# Autodesk Inventor assembly: A103EnsembleChariotCarre
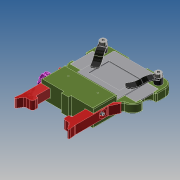
[picture p0: Inventor's stored thumbnail of the model, 180x180]
Saved by Autodesk Inventor 2019 (Build 230136000, 136)
## iProperties
Created: 2016-11-23
Part Number: A103EnsembleChariotCarre
Document SubType Name: Assembly
Designer: serge.amoos
Author: serge.amoos
## Documents named in this file (14)
- Y:\serge.amoos\AAA-FichiersTries\FocalMeasure\A103EnsembleChariotCarre.iam
- Y:\serge.amoos\AAA-FichiersTries\FocalMeasure\P110Poussoir.ipt
- Y:\serge.amoos\AAA-FichiersTries\FocalMeasure\P111Molette.ipt
- Y:\serge.amoos\AAA-FichiersTries\FocalMeasure\P109Ecrou.ipt
- Y:\serge.amoos\AAA-FichiersTries\FocalMeasure\p104levier1.ipt
- Y:\serge.amoos\AAA-FichiersTries\FocalMeasure\p105levier2.ipt
- Y:\serge.amoos\AAA-FichiersTries\FocalMeasure\P103Bielle.ipt
- Y:\serge.amoos\AAA-FichiersTries\FocalMeasure\P113TigeFileteeM3.ipt
- Y:\serge.amoos\AAA-FichiersTries\FocalMeasure\F106EcrouM3.ipt
- Y:\serge.amoos\AAA-FichiersTries\FocalMeasure\F114DiaReseau.ipt
- Y:\serge.amoos\AAA-FichiersTries\FocalMeasure\F115Reseau.ipt
- Y:\serge.amoos\AAA-FichiersTries\FocalMeasure\P124Pince.ipt
- Y:\serge.amoos\AAA-FichiersTries\FocalMeasure\F116VisTcyl6pcM4x12.ipt
- Y:\serge.amoos\AAA-FichiersTries\FocalMeasure\p123chariotcarre.ipt
## Components (17 placed, 13 different names)
1. p123chariotcarre:1 — Mate:1, Mate:2, Mate:3, Flush:1, Tangent:2, Tangent:4, Insert:2, Insert:4, Angle:1, Angle:2, Flush:2, Flush:3, Mate:7, Mate:8, Mate:9, Mate:10, Mate:11, Mate:12, Insert:5, Angle:3, Insert:6, Angle:4
2. P110Poussoir:1 — Insert:2
3. P111Molette:1 — Mate:5, Insert:3, Mate:6, Tangent:5, Flush:4
4. P109Ecrou:1 — Insert:1, Mate:4
5. p104levier1:1 — Mate:3, Tangent:3, Tangent:5, Angle:1, Flush:3
6. p105levier2:1 — Flush:1, Insert:1, Tangent:1, Angle:2, Flush:2
7. P103Bielle:1 — Mate:1, Tangent:3, Tangent:4
8. P103Bielle:2 — Mate:2, Tangent:1, Tangent:2
9. P113TigeFileteeM3:1 — Mate:4, Mate:6, Flush:4
10. F106EcrouM3:1 — Mate:5, Insert:3
11. P110Poussoir:2 — Insert:4
12. F114DiaReseau:1 — Mate:10, Mate:11, Mate:12
13. F115Reseau:1 — Mate:7, Mate:8, Mate:9
14. P124Pince:1 — Insert:5, Angle:3, Insert:8
15. P124Pince:2 — Insert:6, Angle:4, Insert:7
16. F116VisTcyl6pcM4x12:1 — Insert:7
17. F116VisTcyl6pcM4x12:2 — Insert:8
## Relationships (33: Mate 12, Insert 8, Tangent 5, Flush 4, Angle 4)
- Mate:1: p123chariotcarre:1 ↔ P103Bielle:1
- Mate:2: p123chariotcarre:1 ↔ P103Bielle:2
- Mate:3: p123chariotcarre:1 ↔ p104levier1:1
- Flush:1: p123chariotcarre:1 ↔ p105levier2:1
- Insert:1: P109Ecrou:1 ↔ p105levier2:1
- Mate:4: P109Ecrou:1 ↔ P113TigeFileteeM3:1
- Tangent:1: p105levier2:1 ↔ P103Bielle:2
- Tangent:2: p123chariotcarre:1 ↔ P103Bielle:2
- Tangent:3: p104levier1:1 ↔ P103Bielle:1
- Tangent:4: p123chariotcarre:1 ↔ P103Bielle:1
- Insert:2: p123chariotcarre:1 ↔ P110Poussoir:1
- Mate:5: P111Molette:1 ↔ F106EcrouM3:1
- Insert:3: P111Molette:1 ↔ F106EcrouM3:1
- Mate:6: P111Molette:1 ↔ P113TigeFileteeM3:1
- Insert:4: p123chariotcarre:1 ↔ P110Poussoir:2
- Tangent:5: P111Molette:1 ↔ p104levier1:1
- Angle:1 (0 deg): p123chariotcarre:1 ↔ p104levier1:1
- Angle:2 (0 deg): p123chariotcarre:1 ↔ p105levier2:1
- Flush:2 (-1 mm): p123chariotcarre:1 ↔ p105levier2:1
- Flush:3 (1 mm): p123chariotcarre:1 ↔ p104levier1:1
- Flush:4: P111Molette:1 ↔ P113TigeFileteeM3:1
- Mate:7: p123chariotcarre:1 ↔ F115Reseau:1
- Mate:8: p123chariotcarre:1 ↔ F115Reseau:1
- Mate:9: p123chariotcarre:1 ↔ F115Reseau:1
- Mate:10: p123chariotcarre:1 ↔ F114DiaReseau:1
- Mate:11: p123chariotcarre:1 ↔ F114DiaReseau:1
- Mate:12: p123chariotcarre:1 ↔ F114DiaReseau:1
- Insert:5: p123chariotcarre:1 ↔ P124Pince:1
- Angle:3 (-30 deg): p123chariotcarre:1 ↔ P124Pince:1
- Insert:6: p123chariotcarre:1 ↔ P124Pince:2
- Angle:4 (-30 deg): p123chariotcarre:1 ↔ P124Pince:2
- Insert:7: P124Pince:2 ↔ F116VisTcyl6pcM4x12:1
- Insert:8: P124Pince:1 ↔ F116VisTcyl6pcM4x12:2
